# Autodesk Inventor assembly: xDriveShaftBack
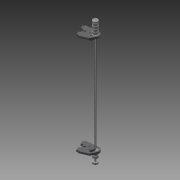
[picture p0: Inventor's stored thumbnail of the model, 180x180]
Saved by Autodesk Inventor 2013 (Build 170138000, 138)
## iProperties
Created: 2015-01-14
Part Number: xDriveShaftBack
Document SubType Name: Assembly
Designer: dzban
Author: dzban
## Documents named in this file (6)
- D:\PIRX\Artisan\OPENSOURCE\SmallPieces\xDriveShaftBack.iam
- D:\PIRX\Artisan\OPENSOURCE\StockComponents\625ZZ_bearing.ipt
- D:\PIRX\Artisan\OPENSOURCE\StockComponents\gt2_20_pulley.ipt
- D:\PIRX\Artisan\OPENSOURCE\SmallPieces\xDriveShaft.ipt
- D:\PIRX\Artisan\OPENSOURCE\SmallPieces\xDriveShaftSupport.ipt
- D:\PIRX\Artisan\OPENSOURCE\SmallPieces\xDriveShaftSupportb.ipt
## Components (12 placed, 5 different names)
1. 625ZZ_bearing:1 — Insert:3, Insert:5
2. 625ZZ_bearing:2 — Insert:4, Insert:6
3. 625ZZ_bearing:3 — Insert:2, Insert:4, Insert:11
4. 625ZZ_bearing:4 — Insert:1, Insert:3
5. gt2_20_pulley:1 — Insert:13
6. gt2_20_pulley:2 — Insert:11, Insert:12
7. gt2_20_pulley:3 — Insert:12
8. xDriveShaft:1 — Insert:1, Insert:2
9. xDriveShaftSupport:1 — Insert:5, Angle:1, Insert:7, Insert:9, Insert:13
10. xDriveShaftSupport:2 — Insert:6, Angle:1, Insert:8, Insert:10
11. xDriveShaftSupportb:1 — Insert:7, Insert:9
12. xDriveShaftSupportb:2 — Insert:8, Insert:10
## Relationships (14: Insert 13, Angle 1)
- Insert:1 (-5 mm): 625ZZ_bearing:4 ↔ xDriveShaft:1
- Insert:2 (-5 mm): 625ZZ_bearing:3 ↔ xDriveShaft:1
- Insert:3 (-38 mm): 625ZZ_bearing:1 ↔ 625ZZ_bearing:4
- Insert:4 (-45 mm): 625ZZ_bearing:2 ↔ 625ZZ_bearing:3
- Insert:5 (-5 mm): 625ZZ_bearing:1 ↔ xDriveShaftSupport:1
- Insert:6 (-5 mm): 625ZZ_bearing:2 ↔ xDriveShaftSupport:2
- Angle:1 (0 deg): xDriveShaftSupport:1 ↔ xDriveShaftSupport:2
- Insert:7: xDriveShaftSupport:1 ↔ xDriveShaftSupportb:1
- Insert:8: xDriveShaftSupport:2 ↔ xDriveShaftSupportb:2
- Insert:9: xDriveShaftSupport:1 ↔ xDriveShaftSupportb:1
- Insert:10: xDriveShaftSupport:2 ↔ xDriveShaftSupportb:2
- Insert:11 (1 mm): 625ZZ_bearing:3 ↔ gt2_20_pulley:2
- Insert:12 (1 mm): gt2_20_pulley:2 ↔ gt2_20_pulley:3
- Insert:13 (1 mm): gt2_20_pulley:1 ↔ xDriveShaftSupport:1
